# Autodesk Inventor assembly: Assembly1
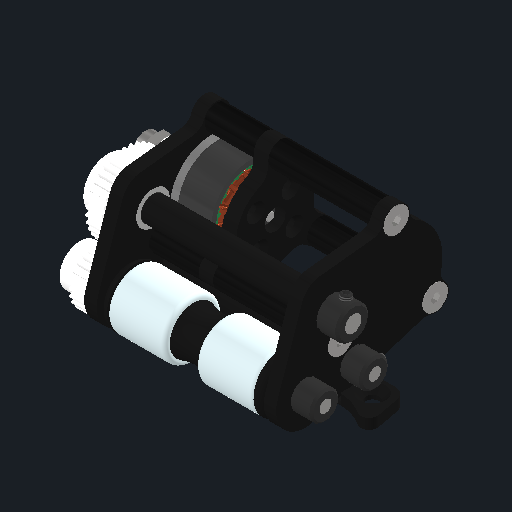
[picture p0: Inventor's stored thumbnail of the model, 512x512]
Saved by Autodesk Inventor 2026.1 (Build 301233020, 233B)
## iProperties
Created: 2026-04-15
Part Number: Assembly1
Document SubType Name: Assembly
Designer: Bahaa
Mass: 570.776 g
Surface Area: 334.489 cm^2
Volume: 26.3276 cm^3
Density: 21.6797 g/cm^3
Author: Bahaa
## Documents named in this file (24)
- C:\Users\Bahaa\Nextcloud2\CAD\25-26\V2\Dribbler\Dribbler V2\Dribbler.iam
- C:\Users\Bahaa\Nextcloud2\CAD\25-26\V2\Dribbler\Dribbler V2\Dribbler Bracket A.ipt
- C:\Users\Bahaa\Nextcloud2\CAD\25-26\V2\Dribbler\Dribbler V2\t-motor-f1507-1.snapshot.1\T-Motor F1507\T-Motor F1507\T-Motor F1507.iam
- C:\Users\Bahaa\Nextcloud2\CAD\25-26\V2\Dribbler\Dribbler V2\Motor Mounting Plate.ipt
- C:\Users\Bahaa\Nextcloud2\CAD\25-26\V2\Dribbler\Dribbler V2\Abstandsbolzen PA6.0 schwarz II Ø6x12 Gewinde M3 durchgehend.ipt
- C:\Users\Bahaa\Nextcloud2\CAD\25-26\V2\Dribbler\Dribbler V2\Miniatur Flanschkugellager MF 63 2RS.ipt
- C:\Users\Bahaa\Nextcloud2\CAD\25-26\V2\Dribbler\Dribbler V2\Miniatur Flanschkugellager MF 74 ZZ.ipt
- C:\Users\Bahaa\Nextcloud2\CAD\25-26\V2\Dribbler\Dribbler V2\Abstandsbolzen PA6.6 schwarz IA Ø6x25 I=M3x10 A=M3x8 o. Freistich.ipt
- C:\Users\Bahaa\Nextcloud2\CAD\25-26\V2\Dribbler\Dribbler V2\MAEDLER_29102000\29102000.ipt
- C:\Users\Bahaa\Nextcloud2\CAD\25-26\V2\Dribbler\Dribbler V2\MAEDLER_29102500\29102500.ipt
- C:\Users\Bahaa\Nextcloud2\CAD\25-26\V2\Dribbler\Dribbler V2\MAEDLER_29103600\29103600.ipt
- C:\Users\Bahaa\Nextcloud2\CAD\25-26\V2\Dribbler\Dribbler V2\Dribbler Bracket B.ipt
- C:\Users\Bahaa\Nextcloud2\CAD\25-26\V2\Dribbler\Dribbler V2\MAEDLER_623890036\AIS2024\623890036.iam
- C:\Users\Bahaa\Nextcloud2\CAD\25-26\V2\Dribbler\Dribbler V2\MAEDLER_623890046\AIS2024\623890046.iam
- C:\Users\Bahaa\Nextcloud2\CAD\25-26\V2\Dribbler\Dribbler V2\M3 Rod.ipt
- C:\Users\Bahaa\Nextcloud2\CAD\25-26\V2\Dribbler\Dribbler V2\M4 Rod.ipt
- C:\Users\Bahaa\Nextcloud2\CAD\25-26\V2\Dribbler\Dribbler V2\M4 Rod Housing.ipt
- C:\Users\Bahaa\Nextcloud2\CAD\25-26\V2\Dribbler\Dribbler V2\Dribbler Roller Seperator.ipt
- C:\Users\Bahaa\Nextcloud2\CAD\25-26\V2\Dribbler\Dribbler V2\Dribbler Roller.ipt
- C:\Users\Bahaa\Documents\Inventor\Content Center Files\R2026\en-US\DIN 7991(2)\DIN 7991 - M3x8.ipt
- C:\Users\Bahaa\Documents\Inventor\Content Center Files\R2026\en-US\DIN 985\DIN 985 - M4.ipt
- C:\Users\Bahaa\Nextcloud2\CAD\25-26\V2\Dribbler\Dribbler V2\t-motor-f1507-1.snapshot.1\T-Motor F1507\T-Motor F1507\Case Motor.ipt
- C:\Users\Bahaa\Nextcloud2\CAD\25-26\V2\Dribbler\Dribbler V2\Dribbler Mount.ipt
- C:\Users\Bahaa\Nextcloud2\CAD\25-26\V2\Dribbler\Dribbler V2\M3 Pivot Rod.ipt
## Components (37 placed, 23 different names)
1. Dribbler Bracket A:1 — Mate:5, Mate:6, Mate:7, Mate:8, Mate:9, Mate:10, Mate:11, Mate:12, Mate:14, Mate:15, Mate:16, Mate:17, Mate:24, Mate:26, Mate:28, Mate:52, Mate:53, Mate:54, Mate:60, Mate:63, Mate:64, Angle:5
2. Dribbler Bracket B:1 — Mate:30, Mate:31, Mate:32, Mate:33, Mate:34, Mate:35, Mate:36, Mate:37, Mate:38, Mate:39, Mate:55, Mate:56, Mate:57, Mate:61, Mate:65, Mate:66
3. Motor Mounting Plate:1 — Mate:1, Mate:2, Mate:3, Mate:5, Mate:6, Mate:13, Mate:18, Mate:19, Mate:20, Mate:21, Mate:22, Mate:23
4. Dribbler Mount:1 — Angle:1, Mate:61, Angle:3, Angle:4, Angle:5, Mate:68
5. DIN 7991 M3x8:1 — Mate:52
6. DIN 7991 M3x8:2 — Mate:53
7. DIN 7991 M3x8:3 — Mate:54
8. DIN 7991 M3x8:4 — Mate:55
9. DIN 7991 M3x8:5 — Mate:56
10. DIN 7991 M3x8:6 — Mate:57
11. DIN 985 - replaced by DIN EN ISO 10511 M4:1 — Insert:1, Rotation:2
12. Abstandsbolzen PA6.0 schwarz II Ø6x12 Gewinde M3 durchgehend:1 — Mate:7, Mate:8
13. Abstandsbolzen PA6.0 schwarz II Ø6x12 Gewinde M3 durchgehend:2 — Mate:9, Mate:10, Mate:13
14. Abstandsbolzen PA6.0 schwarz II Ø6x12 Gewinde M3 durchgehend:3 — Mate:11, Mate:12
15. Abstandsbolzen PA6.6 schwarz IA Ø6x25 I=M3x10 A=M3x8 o. Freistich:1 — Mate:18, Mate:19, Mate:30, Mate:31
16. Abstandsbolzen PA6.6 schwarz IA Ø6x25 I=M3x10 A=M3x8 o. Freistich:2 — Mate:20, Mate:23, Mate:33
17. Abstandsbolzen PA6.6 schwarz IA Ø6x25 I=M3x10 A=M3x8 o. Freistich:3 — Mate:21, Mate:22, Mate:32
18. Miniatur Flanschkugellager MF 63 2RS:1 — Mate:16, Mate:17, Mate:29, Mate:46
19. Miniatur Flanschkugellager MF 63 2RS:2 — Mate:36, Mate:37, Mate:41
20. Miniatur Flanschkugellager MF 74 ZZ:1 — Mate:14, Mate:15, Mate:25, Mate:42
21. Miniatur Flanschkugellager MF 74 ZZ:2 — Mate:34, Mate:35, Mate:40, Mate:45
22. M3 Pivot Rod:1 — Mate:67, Flush:3, Mate:68
23. 623890036:2 [sub-assembly] — Mate:63, Mate:64, Angle:4
24. 623890036:3 [sub-assembly] — Mate:65, Mate:66, Angle:3, Mate:67, Flush:3
25. 623890036:1 [sub-assembly] — Mate:38, Mate:41, Flush:2, Mate:43, Rotation:8
26. 623890046:1 [sub-assembly] — Mate:39, Mate:40, Flush:1
27. M3 Rod:1 — Flush:2, Mate:43, Mate:47
28. M4 Rod:1 — Mate:42, Flush:1, Mate:44
29. M4 Rod Housing:1 — Mate:44, Mate:45
30. 29102000:1 — Mate:26, Insert:1, Mate:58, Rotation:2, Rotation:3, Rotation:4, Rotation:7
31. 29102500:1 — Mate:28, Mate:29, Rotation:1, Rotation:8
32. 29103600:1 — Mate:24, Mate:25, Rotation:1, Rotation:3
33. Dribbler Roller Seperator:1 — Mate:46, Mate:47, Mate:48, Mate:49, Mate:50, Mate:51, Rotation:5, Rotation:6, Rotation:7
34. Dribbler Roller:1 — Mate:48, Mate:49, Rotation:5
35. Dribbler Roller:2 — Mate:50, Mate:51, Rotation:6
36. T-Motor F1507:1 [sub-assembly] — Mate:1, Mate:2, Mate:3, Mate:58, Mate:59
37. Case Motor:1 — Mate:59, Mate:60, Rotation:4
## Relationships (81: Mate 65, RelateRotation 8, Angle 4, Flush 3, Insert 1)
- Mate:1: Motor Mounting Plate:1 ↔ T-Motor F1507:1
- Mate:2: Motor Mounting Plate:1 ↔ T-Motor F1507:1
- Mate:3: Motor Mounting Plate:1 ↔ T-Motor F1507:1
- Mate:5: Dribbler Bracket A:1 ↔ Motor Mounting Plate:1
- Mate:6: Dribbler Bracket A:1 ↔ Motor Mounting Plate:1
- Mate:7: Dribbler Bracket A:1 ↔ Abstandsbolzen PA6.0 schwarz II Ø6x12 Gewinde M3 durchgehend:1
- Mate:8: Dribbler Bracket A:1 ↔ Abstandsbolzen PA6.0 schwarz II Ø6x12 Gewinde M3 durchgehend:1
- Mate:9: Dribbler Bracket A:1 ↔ Abstandsbolzen PA6.0 schwarz II Ø6x12 Gewinde M3 durchgehend:2
- Mate:10: Dribbler Bracket A:1 ↔ Abstandsbolzen PA6.0 schwarz II Ø6x12 Gewinde M3 durchgehend:2
- Mate:11: Dribbler Bracket A:1 ↔ Abstandsbolzen PA6.0 schwarz II Ø6x12 Gewinde M3 durchgehend:3
- Mate:12: Dribbler Bracket A:1 ↔ Abstandsbolzen PA6.0 schwarz II Ø6x12 Gewinde M3 durchgehend:3
- Mate:13: Motor Mounting Plate:1 ↔ Abstandsbolzen PA6.0 schwarz II Ø6x12 Gewinde M3 durchgehend:2
- Mate:14: Dribbler Bracket A:1 ↔ Miniatur Flanschkugellager MF 74 ZZ:1
- Mate:15: Dribbler Bracket A:1 ↔ Miniatur Flanschkugellager MF 74 ZZ:1
- Mate:16: Dribbler Bracket A:1 ↔ Miniatur Flanschkugellager MF 63 2RS:1
- Mate:17: Dribbler Bracket A:1 ↔ Miniatur Flanschkugellager MF 63 2RS:1
- Mate:18: Motor Mounting Plate:1 ↔ Abstandsbolzen PA6.6 schwarz IA Ø6x25 I=M3x10 A=M3x8 o. Freistich:1
- Mate:19: Motor Mounting Plate:1 ↔ Abstandsbolzen PA6.6 schwarz IA Ø6x25 I=M3x10 A=M3x8 o. Freistich:1
- Mate:20: Motor Mounting Plate:1 ↔ Abstandsbolzen PA6.6 schwarz IA Ø6x25 I=M3x10 A=M3x8 o. Freistich:2
- Mate:21: Motor Mounting Plate:1 ↔ Abstandsbolzen PA6.6 schwarz IA Ø6x25 I=M3x10 A=M3x8 o. Freistich:3
- Mate:22: Motor Mounting Plate:1 ↔ Abstandsbolzen PA6.6 schwarz IA Ø6x25 I=M3x10 A=M3x8 o. Freistich:3
- Mate:23: Motor Mounting Plate:1 ↔ Abstandsbolzen PA6.6 schwarz IA Ø6x25 I=M3x10 A=M3x8 o. Freistich:2
- Mate:24: Dribbler Bracket A:1 ↔ 29103600:1
- Mate:25: Miniatur Flanschkugellager MF 74 ZZ:1 ↔ 29103600:1
- Mate:26: Dribbler Bracket A:1 ↔ 29102000:1
- Mate:28: Dribbler Bracket A:1 ↔ 29102500:1
- Mate:29: Miniatur Flanschkugellager MF 63 2RS:1 ↔ 29102500:1
- Mate:30: Dribbler Bracket B:1 ↔ Abstandsbolzen PA6.6 schwarz IA Ø6x25 I=M3x10 A=M3x8 o. Freistich:1
- Mate:31: Dribbler Bracket B:1 ↔ Abstandsbolzen PA6.6 schwarz IA Ø6x25 I=M3x10 A=M3x8 o. Freistich:1
- Mate:32: Dribbler Bracket B:1 ↔ Abstandsbolzen PA6.6 schwarz IA Ø6x25 I=M3x10 A=M3x8 o. Freistich:3
- Mate:33: Dribbler Bracket B:1 ↔ Abstandsbolzen PA6.6 schwarz IA Ø6x25 I=M3x10 A=M3x8 o. Freistich:2
- Mate:34: Dribbler Bracket B:1 ↔ Miniatur Flanschkugellager MF 74 ZZ:2
- Mate:35: Dribbler Bracket B:1 ↔ Miniatur Flanschkugellager MF 74 ZZ:2
- Mate:36: Dribbler Bracket B:1 ↔ Miniatur Flanschkugellager MF 63 2RS:2
- Mate:37: Dribbler Bracket B:1 ↔ Miniatur Flanschkugellager MF 63 2RS:2
- Mate:38: Dribbler Bracket B:1 ↔ 623890036:1
- Mate:39: Dribbler Bracket B:1 ↔ 623890046:1
- Mate:40: Miniatur Flanschkugellager MF 74 ZZ:2 ↔ 623890046:1
- Mate:41: Miniatur Flanschkugellager MF 63 2RS:2 ↔ 623890036:1
- Mate:42: Miniatur Flanschkugellager MF 74 ZZ:1 ↔ M4 Rod:1
- Flush:1: 623890046:1 ↔ M4 Rod:1
- Flush:2: 623890036:1 ↔ M3 Rod:1
- Mate:43: 623890036:1 ↔ M3 Rod:1
- Mate:44: M4 Rod:1 ↔ M4 Rod Housing:1
- Mate:45: Miniatur Flanschkugellager MF 74 ZZ:2 ↔ M4 Rod Housing:1
- Mate:46: Miniatur Flanschkugellager MF 63 2RS:1 ↔ Dribbler Roller Seperator:1
- Mate:47: M3 Rod:1 ↔ Dribbler Roller Seperator:1
- Mate:48: Dribbler Roller Seperator:1 ↔ Dribbler Roller:1
- Mate:49: Dribbler Roller Seperator:1 ↔ Dribbler Roller:1
- Mate:50: Dribbler Roller Seperator:1 ↔ Dribbler Roller:2
- Mate:51: Dribbler Roller Seperator:1 ↔ Dribbler Roller:2
- Mate:52: Dribbler Bracket A:1 ↔ DIN 7991 M3x8:1
- Mate:53: Dribbler Bracket A:1 ↔ DIN 7991 M3x8:2
- Mate:54: Dribbler Bracket A:1 ↔ DIN 7991 M3x8:3
- Mate:55: Dribbler Bracket B:1 ↔ DIN 7991 M3x8:4
- Mate:56: Dribbler Bracket B:1 ↔ DIN 7991 M3x8:5
- Mate:57: Dribbler Bracket B:1 ↔ DIN 7991 M3x8:6
- Insert:1: DIN 985 - replaced by DIN EN ISO 10511 M4:1 ↔ 29102000:1
- Mate:58: 29102000:1 ↔ T-Motor F1507:1
- Rotation:1 [RelateRotation] (1.44 ul): 29102500:1 ↔ 29103600:1
- Rotation:2 [RelateRotation] (1 ul): DIN 985 - replaced by DIN EN ISO 10511 M4:1 ↔ 29102000:1
- Rotation:3 [RelateRotation] (0.5556 ul): 29102000:1 ↔ 29103600:1
- Mate:59: T-Motor F1507:1 ↔ Case Motor:1
- Mate:60: Dribbler Bracket A:1 ↔ Case Motor:1
- Rotation:4 [RelateRotation] (1 ul): 29102000:1 ↔ Case Motor:1
- Rotation:5 [RelateRotation] (1 ul): Dribbler Roller Seperator:1 ↔ Dribbler Roller:1
- Rotation:6 [RelateRotation] (1 ul): Dribbler Roller Seperator:1 ↔ Dribbler Roller:2
- Rotation:7 [RelateRotation] (1 ul): 29102000:1 ↔ Dribbler Roller Seperator:1
- Angle:1 (0 deg): Dribbler Mount:1
- Mate:61 (0.125 mm): Dribbler Bracket B:1 ↔ Dribbler Mount:1
- Mate:63: Dribbler Bracket A:1 ↔ 623890036:2
- Mate:64: Dribbler Bracket A:1 ↔ 623890036:2
- Mate:65: Dribbler Bracket B:1 ↔ 623890036:3
- Mate:66: Dribbler Bracket B:1 ↔ 623890036:3
- Angle:3 (270 deg): Dribbler Mount:1 ↔ 623890036:3
- Angle:4 (90 deg): Dribbler Mount:1 ↔ 623890036:2
- Mate:67: M3 Pivot Rod:1 ↔ 623890036:3
- Flush:3: M3 Pivot Rod:1 ↔ 623890036:3
- Angle:5 (162.5 deg): Dribbler Bracket A:1 ↔ Dribbler Mount:1
- Rotation:8 [RelateRotation] (1.429 ul): 623890036:1 ↔ 29102500:1
- Mate:68: Dribbler Mount:1 ↔ M3 Pivot Rod:1
